# Autodesk Inventor assembly: hcsr04
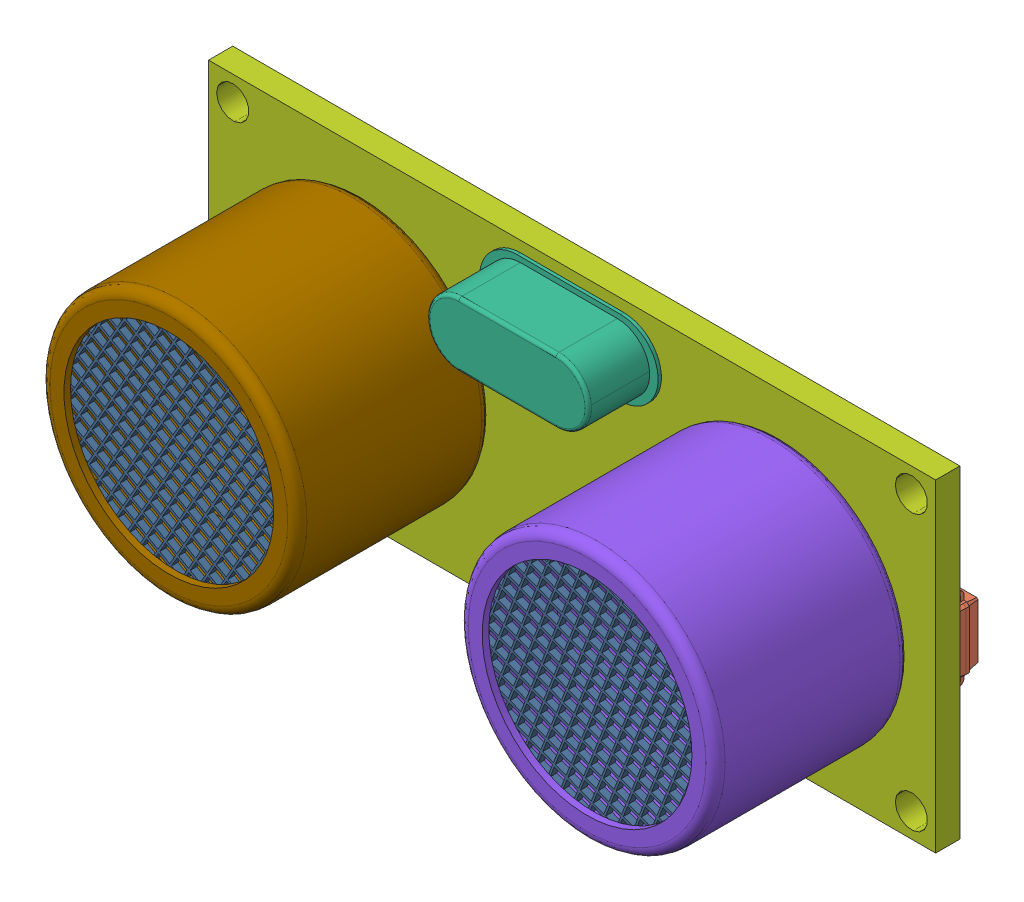
[picture p0: shaded view drawn from the shape stored in the file]
Saved by Autodesk Inventor 2021 (Build 250183000, 183)
## iProperties
Company: Unknown
Created: 2018-10-29
Part Number: hcsr04
Description: Unknown
Document SubType Name: Assembly
Designer: User
Sending System: DEX
Preprocessor: ST-DEVELOPER v16.7
Title: HC-SR04
Author: Unknown
## Documents named in this file (10)
- D:\SynologyDrive\tcodev\tco-cad\common\hcsr04\hcsr04.iam
- D:\SynologyDrive\tcodev\tco-cad\common\hcsr04\Transducer.ipt
- D:\SynologyDrive\tcodev\tco-cad\common\hcsr04\Mesh.ipt
- D:\SynologyDrive\tcodev\tco-cad\common\hcsr04\Board.ipt
- D:\SynologyDrive\tcodev\tco-cad\common\kicad_packages_3d\SOIC-16_3.9x9.9mm_P1.27mm.ipt
- D:\SynologyDrive\tcodev\tco-cad\common\kicad_packages_3d\SOIC-14_3.9x8.7mm_P1.27mm.ipt
- D:\SynologyDrive\tcodev\tco-cad\common\kicad_packages_3d\C_0603_1608Metric.ipt
- D:\SynologyDrive\tcodev\tco-cad\common\kicad_packages_3d\R_0603_1608Metric.ipt
- D:\SynologyDrive\tcodev\tco-cad\common\kicad_packages_3d\PinHeader_1x04_P2.54mm_Horizontal.ipt
- D:\SynologyDrive\tcodev\tco-cad\common\kicad_packages_3d\Crystal_HC49-4H_Vertical.ipt
## Components (21 placed, 9 different names)
1. Board — Mate:4, Angle:3, Mate:5, Mate:6, Angle:4, Angle:5, Mate:7, Mate:8, Mate:9, Mate:10, Mate:11, Mate:12, Mate:13, Mate:14, Mate:15, Rigid:1, Rigid:2
2. Crystal_HC49-4H_Vertical:1 — Rigid:2
3. Transducer — Mate:16, Mate:17, Mate:18, Mate:19
4. Mesh — Mate:16, Mate:19
5. Mesh:1 — Mate:17, Mate:18
6. SOIC-16_3.9x9.9mm_P1.27mm:3 — Mate:4, Angle:3
7. SOIC-14_3.9x8.7mm_P1.27mm:1 — Mate:5, Angle:4
8. SOIC-14_3.9x8.7mm_P1.27mm:2 — Mate:6, Angle:5
9. C_0603_1608Metric:4 — Mate:9, Flush:3, Flush:8
10. C_0603_1608Metric:5 — Mate:10, Flush:3, Flush:4, Flush:8, Flush:9
11. C_0603_1608Metric:6 — Mate:11, Flush:5, Flush:6, Flush:10, Flush:11
12. R_0603_1608Metric:4 — Mate:12, Flush:4, Flush:5, Flush:9, Flush:10
13. R_0603_1608Metric:5 — Mate:13, Flush:6, Flush:7, Flush:11, Flush:12
14. R_0603_1608Metric:6 — Mate:14, Flush:7, Flush:12
15. PinHeader_1x04_P2.54mm_Horizontal:1 — Mate:15, Rigid:1
16. R_0603_1608Metric:1 — Mate:8, Flush:2
17. R_0603_1608Metric:2
18. R_0603_1608Metric:3
19. C_0603_1608Metric:1 — Mate:7, Flush:2
20. C_0603_1608Metric:2
21. C_0603_1608Metric:3
## Component patterns: (3 elements, first: R_0603_1608Metric:1), (3 elements, first: C_0603_1608Metric:1)
## Relationships (32: Mate 16, Flush 11, Angle 3, WeldJoint 2)
- Mate:4: Board ↔ SOIC-16_3.9x9.9mm_P1.27mm:3
- Angle:3 (0 deg): Board ↔ SOIC-16_3.9x9.9mm_P1.27mm:3
- Mate:5: Board ↔ SOIC-14_3.9x8.7mm_P1.27mm:1
- Mate:6: Board ↔ SOIC-14_3.9x8.7mm_P1.27mm:2
- Angle:4 (0 deg): Board ↔ SOIC-14_3.9x8.7mm_P1.27mm:1
- Angle:5 (0 deg): Board ↔ SOIC-14_3.9x8.7mm_P1.27mm:2
- Mate:7: Board ↔ C_0603_1608Metric:1
- Mate:8: Board ↔ R_0603_1608Metric:1
- Flush:2: R_0603_1608Metric:1 ↔ C_0603_1608Metric:1
- Mate:9: Board ↔ C_0603_1608Metric:4
- Mate:10: Board ↔ C_0603_1608Metric:5
- Mate:11: Board ↔ C_0603_1608Metric:6
- Mate:12: Board ↔ R_0603_1608Metric:4
- Mate:13: Board ↔ R_0603_1608Metric:5
- Mate:14: Board ↔ R_0603_1608Metric:6
- Flush:3: C_0603_1608Metric:4 ↔ C_0603_1608Metric:5
- Flush:4: C_0603_1608Metric:5 ↔ R_0603_1608Metric:4
- Flush:5: C_0603_1608Metric:6 ↔ R_0603_1608Metric:4
- Flush:6: C_0603_1608Metric:6 ↔ R_0603_1608Metric:5
- Flush:7: R_0603_1608Metric:5 ↔ R_0603_1608Metric:6
- Flush:8 (2.15 mm): C_0603_1608Metric:4 ↔ C_0603_1608Metric:5
- Flush:9 (2.15 mm): C_0603_1608Metric:5 ↔ R_0603_1608Metric:4
- Flush:10 (2.15 mm): C_0603_1608Metric:6 ↔ R_0603_1608Metric:4
- Flush:11 (2.15 mm): C_0603_1608Metric:6 ↔ R_0603_1608Metric:5
- Flush:12 (2.15 mm): R_0603_1608Metric:5 ↔ R_0603_1608Metric:6
- Mate:15: Board ↔ PinHeader_1x04_P2.54mm_Horizontal:1
- Rigid:1 [WeldJoint] (-3 mm): Board ↔ PinHeader_1x04_P2.54mm_Horizontal:1
- Rigid:2 [WeldJoint] (-3 mm): Board ↔ Crystal_HC49-4H_Vertical:1
- Mate:16: Transducer ↔ Mesh
- Mate:17: Transducer ↔ Mesh:1
- Mate:18: Transducer ↔ Mesh:1
- Mate:19: Transducer ↔ Mesh
